# Autodesk Inventor assembly: FullApparatus
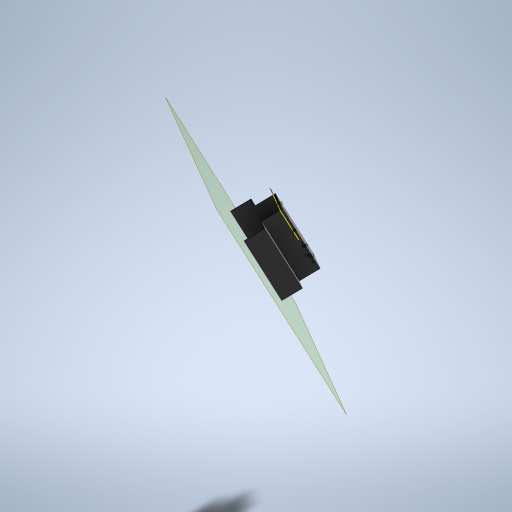
[picture p0: Inventor's stored thumbnail of the model, 512x512]
Saved by Autodesk Inventor 2023 (Build 270158000, 158)
## iProperties
Created: 2019-09-17
Part Number: FullApparatus
Document SubType Name: Assembly
Designer: Knowblesse
Author: Knowblesse
## Documents named in this file (4)
- C:\VCF\Lobster\Apparatus\FullApparatus.iam
- C:\VCF\Lobster\Apparatus\Arena\Main.ipt
- C:\VCF\Lobster\Apparatus\Robot\Motor_Panel.iam
- C:\VCF\Lobster\Apparatus\Arena\IRLight.ipt
## Components (3 placed, 3 different names)
1. Main:1 — 강체:1, 강체:2, 메이트:1, 메이트:2, Flush:1
2. Motor_Panel:1 [sub-assembly] — 강체:1
3. IRLight:1 — 강체:2
## Relationships (5: WeldJoint 2, Mate 2, Flush 1)
- 강체:1 [WeldJoint]: Main:1 ↔ Motor_Panel:1
- 강체:2 [WeldJoint]: Main:1 ↔ IRLight:1
- 메이트:1 [Mate]: Main:1
- 메이트:2 [Mate]: Main:1
- Flush:1 (150 mm): Main:1
